# Autodesk Inventor assembly: Lower skin assembly
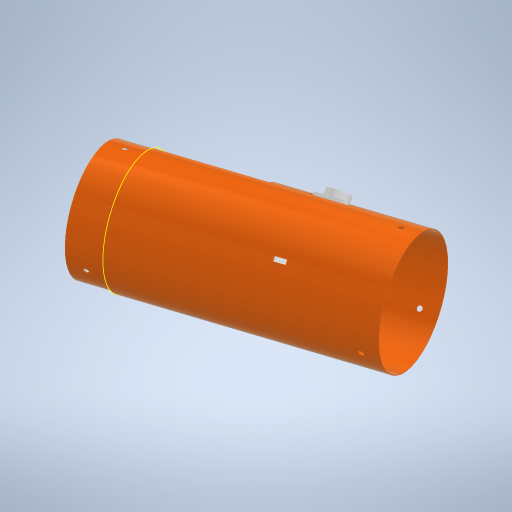
[picture p0: Inventor's stored thumbnail of the model, 512x512]
Saved by Autodesk Inventor 2024 (Build 280153000, 153)
## iProperties
Created: 2024-04-27
Part Number: Lower skin assembly
Document SubType Name: Assembly
Designer: auror
Author: auror
## Documents named in this file (5)
- C:\Users\auror\Documents\TU Delft\DARE\Git\Scrambler-2-CAD\Autodesk\Lower skin assembly.iam
- C:\Users\auror\Documents\TU Delft\DARE\Git\Scrambler-2-CAD\Autodesk\Electronics Door.ipt
- C:\Users\auror\Documents\TU Delft\DARE\Git\Scrambler-2-CAD\Autodesk\Lower skin.ipt
- C:\Users\auror\Documents\TU Delft\DARE\Git\Scrambler-2-CAD\Autodesk\Electronic Assembly.iam
- C:\Users\auror\Documents\TU Delft\DARE\Scrambler-II\Button.ipt
## Components (5 placed, 4 different names)
1. Electronics Door:1 — Mate:24
2. Lower skin:1 — Mate:24, Mate:25, Mate:26, Mate:27, Mate:28, Mate:29, Mate:30, Angle:1, Angle:2
3. Electronic Assembly:1 [sub-assembly] — Mate:25, Mate:26
4. Button:1 — Mate:29, Mate:30, Angle:1
5. Button:2 — Mate:27, Mate:28, Angle:2
## Relationships (9: Mate 7, Angle 2)
- Mate:24: Electronics Door:1 ↔ Lower skin:1
- Mate:25: Lower skin:1 ↔ Electronic Assembly:1
- Mate:26: Lower skin:1 ↔ Electronic Assembly:1
- Mate:27: Lower skin:1 ↔ Button:2
- Mate:28: Lower skin:1 ↔ Button:2
- Mate:29: Lower skin:1 ↔ Button:1
- Mate:30: Lower skin:1 ↔ Button:1
- Angle:1 (0 deg): Lower skin:1 ↔ Button:1
- Angle:2 (0 deg): Lower skin:1 ↔ Button:2
